# Autodesk Inventor assembly: Montagem Gabinete
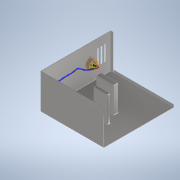
[picture p0: Inventor's stored thumbnail of the model, 180x180]
Saved by Autodesk Inventor 2021 (Build 250183000, 183)
## iProperties
Created: 2021-05-27
Part Number: Montagem Gabinete
Document SubType Name: Assembly
Designer: rubia
Author: rubia
## Documents named in this file (5)
- C:\Users\rubia\OneDrive\Documentos\Inventor\Rubia_ASR11\Montagem Gabinete.iam
- C:\Users\rubia\OneDrive\Documentos\Inventor\Rubia_ASR11\Conector1.ipt
- C:\Users\rubia\OneDrive\Documentos\Inventor\Rubia_ASR11\Conector2.ipt
- C:\Users\rubia\OneDrive\Documentos\Inventor\Rubia_ASR11\Gabinete.ipt
- C:\Users\rubia\OneDrive\Documentos\Inventor\Rubia_ASR11\Montagem Gabinete.Fiação1.iam
## Components (4 placed, 4 different names)
1. Conector1:1 — Coincidente:1, Coincidente:2, Coincidente:3
2. Conector2:1 — Coincidente:4, Coincidente:5, Coincidente:6
3. Gabinete:1 — Coincidente:1, Coincidente:2, Coincidente:3, Coincidente:4, Coincidente:5, Coincidente:6
4. Fiação1 [sub-assembly]
## Relationships (6: Mate 6)
- Coincidente:1 [Mate]: Conector1:1 ↔ Gabinete:1
- Coincidente:2 [Mate]: Conector1:1 ↔ Gabinete:1
- Coincidente:3 [Mate]: Conector1:1 ↔ Gabinete:1
- Coincidente:4 [Mate]: Conector2:1 ↔ Gabinete:1
- Coincidente:5 [Mate]: Conector2:1 ↔ Gabinete:1
- Coincidente:6 [Mate]: Conector2:1 ↔ Gabinete:1
